# Autodesk Inventor assembly: 24x32 Side Rail Sub mirror
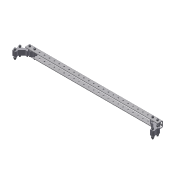
[picture p0: Inventor's stored thumbnail of the model, 180x180]
Saved by Autodesk Inventor 2013 (Build 170138000, 138)
## iProperties
Created: 2013-01-06
Part Number: 24x32 Side Rail Sub mirror
Document SubType Name: Assembly
Designer: Nemo
Author: Nemo
## Documents named in this file (4)
- \\lmss\STUDENTS\Robotics\CAD Files\COTS Parts\Kit Frame - AndyMark\Components\26x30 Side Rail Sub mirror.iam
- \\lmss\STUDENTS\Robotics\CAD Files\COTS Parts\Kit Frame - AndyMark\Components\CornerConnectAssyLeft.iam
- \\lmss\STUDENTS\Robotics\CAD Files\COTS Parts\Kit Frame - AndyMark\Components\CornerConnectAssyRight.iam
- \\lmss\STUDENTS\Robotics\CAD Files\COTS Parts\Kit Frame - AndyMark\Components\C Channel - Side 26x30.ipt
## Components (3 placed, 3 different names)
1. C Channel - Cut-01:2 — Insert:1, Mate:1, Insert:2, Mate:2
2. CornerConnectAssyLeft:1 [sub-assembly] — Insert:2, Mate:2
3. CornerConnectAssyRight:1 [sub-assembly] — Insert:1, Mate:1
## Relationships (4: Insert 2, Mate 2)
- Insert:1: C Channel - Cut-01:2 ↔ CornerConnectAssyRight:1
- Mate:1: C Channel - Cut-01:2 ↔ CornerConnectAssyRight:1
- Insert:2: C Channel - Cut-01:2 ↔ CornerConnectAssyLeft:1
- Mate:2: C Channel - Cut-01:2 ↔ CornerConnectAssyLeft:1
